# Autodesk Inventor assembly: LED Bar
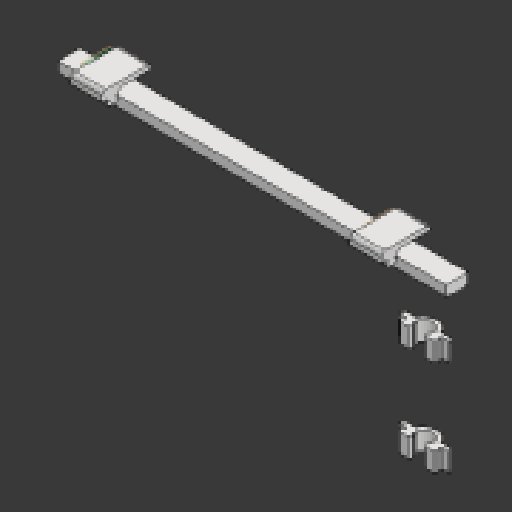
[picture p0: Inventor's stored thumbnail of the model, 512x512]
Saved by Autodesk Inventor 2023 (Build 270158000, 158)
## iProperties
Created: 2023-01-05
Part Number: LED Bar
Document SubType Name: Assembly
Designer: alber
Author: alber
## Documents named in this file (6)
- C:\Users\alber\Desktop\Files\Ender3-Upgrade\CAD\LED Bar.iam
- C:\Users\alber\Desktop\Files\Ender3-Upgrade\CAD\Led Light.ipt
- C:\Users\alber\Desktop\Files\Ender3-Upgrade\CAD\LED Holder.ipt
- C:\Users\alber\Desktop\Files\Ender3-Upgrade\CAD\LED Holder Magnetic.ipt
- C:\Users\alber\Desktop\Files\Ender3-Upgrade\CAD\Camera Wire Clip.ipt
- C:\Users\alber\Desktop\Files\Ender3-Upgrade\CAD\USB Light Cable.ipt
## Components (8 placed, 5 different names)
1. Led Light:1 — Flush:5, Flush:6
2. LED Holder:1
3. LED Holder Magnetic:1
4. LED Holder Magnetic:2
5. LED Holder:2
6. Camera Wire Clip:1
7. Camera Wire Clip:2
8. USB Light Cable:1 — Flush:5, Flush:6
## Relationships (7: Flush 6, Mate 1)
- [Flush]: LED Holder:1 ↔ LED Holder Magnetic:1
- [Flush]: LED Holder:1 ↔ LED Holder Magnetic:1
- [Flush]: LED Holder Magnetic:2 ↔ LED Holder:2
- [Flush]: LED Holder:1 ↔ LED Holder:2
- [Mate]: LED Holder Magnetic:2 ↔ LED Holder:2
- Flush:5: Led Light:1 ↔ USB Light Cable:1
- Flush:6: Led Light:1 ↔ USB Light Cable:1
## Named parameters: d2_d4 = 0 mm
